# Autodesk Inventor assembly: Table
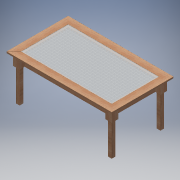
[picture p0: Inventor's stored thumbnail of the model, 180x180]
Saved by Autodesk Inventor 2016 (Build 200138000, 138)
## iProperties
Created: 2016-02-08
Part Number: Table
Document SubType Name: Assembly
Designer: ron
Mass: 50986 g
Surface Area: 141310 cm^2
Volume: 60602.2 cm^3
Density: 0.841322 g/cm^3
Author: ron
## Documents named in this file (20)
- C:\Users\ron\Documents\GitHub\CoffeeTableCAD\Table.iam
- C:\Users\ron\Documents\GitHub\CoffeeTableCAD\Parts\LedBoard.ipt
- C:\Users\ron\Documents\GitHub\CoffeeTableCAD\Parts\Acrylitep95.ipt
- C:\Users\ron\Documents\GitHub\CoffeeTableCAD\Parts\LegStandard.ipt
- C:\Users\ron\Documents\GitHub\CoffeeTableCAD\Parts\Glass.ipt
- C:\Users\ron\Documents\GitHub\CoffeeTableCAD\Parts\LegOutlet.ipt
- C:\Users\ron\Documents\GitHub\CoffeeTableCAD\Parts\Bottom.ipt
- C:\Users\ron\Documents\GitHub\CoffeeTableCAD\Parts\PowerSupply.ipt
- C:\Users\ron\Documents\GitHub\CoffeeTableCAD\Parts\Magnet.ipt
- C:\Users\ron\Documents\GitHub\CoffeeTableCAD\Parts\DividerWidthPlastic.ipt
- C:\Users\ron\Documents\GitHub\CoffeeTableCAD\Parts\DividerLengthPlastic.ipt
- C:\Users\ron\Documents\GitHub\CoffeeTableCAD\Parts\SkinnySideWidth.ipt
- C:\Users\ron\Documents\GitHub\CoffeeTableCAD\Parts\SkinnySideLength.ipt
- C:\Users\ron\Documents\GitHub\CoffeeTableCAD\Parts\SkirtLength.ipt
- C:\Users\ron\Documents\GitHub\CoffeeTableCAD\Parts\SkirtWidth.ipt
- C:\Users\ron\Documents\GitHub\CoffeeTableCAD\Parts\LegHolder.ipt
- C:\Users\ron\Documents\GitHub\CoffeeTableCAD\Parts\SkinnySideWidthOutlet.ipt
- C:\Users\ron\Documents\GitHub\CoffeeTableCAD\Parts\SkinnySideLengthPower.ipt
- C:\Users\ron\Documents\GitHub\CoffeeTableCAD\Parts\LegHolderOutlet.ipt
- C:\Users\ron\Documents\GitHub\CoffeeTableCAD\Parts\SupportWedge.ipt
## Components (77 placed, 19 different names)
1. LedBoard:1 — Flush:127, Flush:128, Mate:93, Mate:94, Flush:138, Flush:139, Flush:140, Flush:141, Flush:143, Flush:144, Flush:146, Flush:147, Flush:149, Flush:150, Flush:152, Flush:153, Flush:155, Flush:156, Flush:158, Flush:159, Flush:161, Flush:162, Flush:164, Flush:165, Flush:167, Flush:168, Flush:170, Flush:171, Flush:173, Flush:174, Flush:176, Flush:177, Flush:179, Flush:180, Flush:182, Flush:183, Flush:185, Flush:186, Flush:188, Flush:189, Flush:191, Flush:192, Flush:194, Flush:195, Flush:197, Flush:198, Flush:200, Flush:201, Flush:203, Flush:204, Flush:206, Flush:207, Flush:209, Flush:210, Flush:212, Flush:213, Flush:215, Flush:216, Flush:218, Flush:220, Flush:221, Flush:223, Flush:224, Flush:226, Flush:227, Flush:229, Mate:95, Flush:230, Flush:231, Mate:96, Flush:232, Mate:97, Flush:234, Mate:98, Flush:236, Mate:99, Flush:238, Mate:100, Flush:240, Mate:101, Flush:242, Mate:102, Flush:244, Mate:103, Flush:246, Mate:104, Flush:249, Mate:105, Flush:251, Mate:106, Flush:253, Mate:107, Flush:255, Mate:108, Flush:257, Mate:109, Flush:259, Mate:113, Mate:115, Mate:128, Mate:129, Mate:130, Mate:131, Mate:139, Mate:142, Mate:144
2. Acrylitep95:1 — Flush:127, Flush:128, Mate:20, Flush:129, Flush:130, Mate:93, Mate:117, Mate:119, Mate:122, Mate:125
3. LegStandard:1 — Mate:89, Mate:90, Flush:136, Mate:135, Mate:136, Mate:137
4. LegStandard:2 — Mate:91, Mate:92, Flush:137, Mate:148, Mate:149, Mate:150
5. LegStandard:3 — Mate:85, Mate:86, Flush:134, Mate:151, Mate:152, Mate:153
6. LegOutlet:1 — Mate:87, Mate:88, Flush:135, Mate:138, Mate:145, Mate:146, Mate:147
7. Glass:1 — Mate:20, Flush:129, Flush:130, Mate:118, Mate:121, Mate:124
8. Bottom:1 — Flush:131, Flush:132, Mate:167, Mate:168, Mate:169, Mate:170
9. PowerSupply:1 — Flush:131, Flush:132, Mate:170
10. Magnet:3 — Mate:85, Mate:86, Flush:134
11. Magnet:4 — Mate:89, Mate:90, Flush:136
12. Magnet:5 — Mate:87, Mate:88, Flush:135
13. Magnet:6 — Mate:91, Mate:92, Flush:137
14. DividerWidthPlastic:1 — Flush:161, Flush:162, Flush:163, Flush:166
15. DividerWidthPlastic:2 — Flush:167, Flush:168, Flush:169, Flush:172
16. DividerWidthPlastic:3 — Flush:176, Flush:177, Flush:178, Flush:181
17. DividerWidthPlastic:4 — Flush:215, Flush:216, Flush:217, Flush:219
18. DividerWidthPlastic:6 — Flush:170, Flush:171, Flush:172, Flush:175
19. DividerWidthPlastic:7 — Flush:164, Flush:165, Flush:166, Flush:169
20. DividerWidthPlastic:8 — Flush:155, Flush:156, Flush:157, Flush:160
21. DividerWidthPlastic:9 — Flush:158, Flush:159, Flush:160, Flush:163
22. DividerWidthPlastic:10 — Flush:188, Flush:189, Flush:190, Flush:193
23. DividerWidthPlastic:11 — Flush:212, Flush:213, Flush:214, Flush:217
24. DividerWidthPlastic:12 — Flush:218, Flush:219, Flush:220, Flush:222
25. DividerWidthPlastic:13 — Flush:185, Flush:186, Flush:187, Flush:190
26. DividerWidthPlastic:14 — Flush:182, Flush:183, Flush:184, Flush:187
27. DividerWidthPlastic:15 — Flush:179, Flush:180, Flush:181, Flush:184
28. DividerWidthPlastic:16 — Flush:200, Flush:201, Flush:202, Flush:205
29. DividerWidthPlastic:17 — Flush:194, Flush:195, Flush:196, Flush:199
30. DividerWidthPlastic:18 — Flush:191, Flush:192, Flush:193, Flush:196
31. DividerWidthPlastic:19 — Flush:197, Flush:198, Flush:199, Flush:202
32. DividerWidthPlastic:20 — Flush:209, Flush:210, Flush:211, Flush:214
33. DividerWidthPlastic:21 — Mate:94, Flush:138, Flush:139, Flush:142
34. DividerWidthPlastic:22 — Flush:149, Flush:150, Flush:151, Flush:154
35. DividerWidthPlastic:23 — Flush:206, Flush:207, Flush:208, Flush:211
36. DividerWidthPlastic:24 — Flush:140, Flush:141, Flush:142, Flush:145, Mate:120
37. DividerWidthPlastic:25 — Flush:203, Flush:204, Flush:205, Flush:208
38. DividerWidthPlastic:26 — Flush:143, Flush:144, Flush:145, Flush:148
39. DividerWidthPlastic:27 — Flush:146, Flush:147, Flush:148, Flush:151
40. DividerWidthPlastic:28 — Flush:152, Flush:153, Flush:154, Flush:157
41. DividerWidthPlastic:29 — Flush:221, Flush:222, Flush:223, Flush:225
42. DividerWidthPlastic:30 — Flush:224, Flush:225, Flush:226, Flush:228
43. DividerWidthPlastic:31 — Flush:227, Flush:228, Flush:229
44. DividerWidthPlastic:32 — Flush:173, Flush:174, Flush:175, Flush:178
45. DividerLengthPlastic:1 — Mate:95, Flush:230, Flush:231, Flush:233
46. DividerLengthPlastic:2 — Mate:98, Flush:236, Flush:237, Flush:239
47. DividerLengthPlastic:3 — Mate:99, Flush:238, Flush:239, Flush:241
48. DividerLengthPlastic:4 — Mate:104, Flush:248, Flush:249, Flush:250
49. DividerLengthPlastic:5 — Mate:107, Flush:254, Flush:255, Flush:256
50. DividerLengthPlastic:7 — Mate:109, Flush:258, Flush:259
51. DividerLengthPlastic:8 — Mate:105, Flush:250, Flush:251, Flush:252
52. DividerLengthPlastic:9 — Mate:103, Flush:246, Flush:247, Flush:248
53. DividerLengthPlastic:10 — Mate:101, Flush:242, Flush:243, Flush:245
54. DividerLengthPlastic:11 — Mate:97, Flush:234, Flush:235, Flush:237
55. DividerLengthPlastic:12 — Mate:96, Flush:232, Flush:233, Flush:235
56. DividerLengthPlastic:13 — Mate:100, Flush:240, Flush:241, Flush:243, Mate:141
57. DividerLengthPlastic:14 — Mate:102, Flush:244, Flush:245, Flush:247
58. DividerLengthPlastic:15 — Mate:106, Flush:252, Flush:253, Flush:254, Mate:123
59. DividerLengthPlastic:17 — Mate:108, Flush:256, Flush:257, Flush:258, Mate:116
60. SkinnySideWidth:1 — Mate:113, Mate:115, Mate:128, Mate:134, Mate:143, Mate:152, Mate:156, Flush:260, Flush:261, Mate:167, Mate:169
61. SkirtLength:1 — Mate:119, Mate:120, Mate:121, Mate:132, Mate:148, Mate:171, Mate:180, Mate:181, Mate:182
62. SkirtLength:2 — Mate:125, Mate:126, Mate:127, Mate:151, Mate:154, Mate:174, Mate:175, Mate:177, Mate:179
63. SkirtWidth:1 — Mate:116, Mate:117, Mate:118, Mate:127, Mate:135, Mate:176
64. SkirtWidth:2 — Mate:122, Mate:123, Mate:124, Mate:126, Mate:138, Mate:145, Mate:147, Mate:150, Mate:157, Mate:160, Mate:172, Mate:173, Mate:178
65. SkinnySideLength:1 — Mate:129, Mate:130, Mate:131, Mate:133, Mate:140, Mate:149, Mate:159, Mate:166
66. SkinnySideWidthOutlet:1 — Mate:139, Mate:140, Mate:141, Mate:158, Mate:162, Mate:164, Mate:165
67. SkinnySideLengthPower:1 — Mate:142, Mate:143, Mate:144, Mate:146, Mate:153, Mate:155, Mate:161, Mate:163, Mate:168
68. LegHolder:1 — Mate:132, Mate:133, Mate:134, Mate:136, Mate:137
69. LegHolder:2 — Mate:154, Mate:155, Mate:156
70. LegHolder:3 — Mate:157, Mate:158, Mate:159
71. LegHolderOutlet:1 — Mate:160, Mate:161, Mate:162
72. SupportWedge:1 — Flush:260, Mate:163, Mate:164
73. SupportWedge:2 — Flush:261, Mate:165, Mate:166
74. Magnet:7 — Mate:180, Mate:181, Mate:182
75. Magnet:8 — Mate:174, Mate:175, Mate:176
76. Magnet:9 — Mate:171, Mate:172, Mate:173
77. Magnet:10 — Mate:177, Mate:178, Mate:179
## Relationships (229: Flush 134, Mate 95)
- Flush:127 (-25.4 mm): LedBoard:1 ↔ Acrylitep95:1
- Flush:128 (-25.4 mm): LedBoard:1 ↔ Acrylitep95:1
- Mate:20: Acrylitep95:1 ↔ Glass:1
- Flush:129: Acrylitep95:1 ↔ Glass:1
- Flush:130: Acrylitep95:1 ↔ Glass:1
- Flush:131 (50.8 mm): Bottom:1 ↔ PowerSupply:1
- Flush:132 (50.8 mm): Bottom:1 ↔ PowerSupply:1
- Mate:85: LegStandard:3 ↔ Magnet:3
- Mate:86: LegStandard:3 ↔ Magnet:3
- Flush:134: LegStandard:3 ↔ Magnet:3
- Mate:87: LegOutlet:1 ↔ Magnet:5
- Mate:88: LegOutlet:1 ↔ Magnet:5
- Flush:135: LegOutlet:1 ↔ Magnet:5
- Mate:89: LegStandard:1 ↔ Magnet:4
- Mate:90: LegStandard:1 ↔ Magnet:4
- Flush:136: LegStandard:1 ↔ Magnet:4
- Mate:91: LegStandard:2 ↔ Magnet:6
- Mate:92: LegStandard:2 ↔ Magnet:6
- Flush:137: LegStandard:2 ↔ Magnet:6
- Mate:93 (50.8 mm): LedBoard:1 ↔ Acrylitep95:1
- Mate:94: LedBoard:1 ↔ DividerWidthPlastic:21
- Flush:138: LedBoard:1 ↔ DividerWidthPlastic:21
- Flush:139 (36.5125 mm): LedBoard:1 ↔ DividerWidthPlastic:21
- Flush:140 (-50.8 mm): LedBoard:1 ↔ DividerWidthPlastic:24
- Flush:141: LedBoard:1 ↔ DividerWidthPlastic:24
- Flush:142 (38.1 mm): DividerWidthPlastic:21 ↔ DividerWidthPlastic:24
- Flush:143 (-50.8 mm): LedBoard:1 ↔ DividerWidthPlastic:26
- Flush:144: LedBoard:1 ↔ DividerWidthPlastic:26
- Flush:145 (38.1 mm): DividerWidthPlastic:24 ↔ DividerWidthPlastic:26
- Flush:146 (-50.8 mm): LedBoard:1 ↔ DividerWidthPlastic:27
- Flush:147: LedBoard:1 ↔ DividerWidthPlastic:27
- Flush:148 (38.1 mm): DividerWidthPlastic:26 ↔ DividerWidthPlastic:27
- Flush:149 (-50.8 mm): LedBoard:1 ↔ DividerWidthPlastic:22
- Flush:150: LedBoard:1 ↔ DividerWidthPlastic:22
- Flush:151 (38.1 mm): DividerWidthPlastic:22 ↔ DividerWidthPlastic:27
- Flush:152 (-50.8 mm): LedBoard:1 ↔ DividerWidthPlastic:28
- Flush:153: LedBoard:1 ↔ DividerWidthPlastic:28
- Flush:154 (38.1 mm): DividerWidthPlastic:22 ↔ DividerWidthPlastic:28
- Flush:155 (-50.8 mm): LedBoard:1 ↔ DividerWidthPlastic:8
- Flush:156: LedBoard:1 ↔ DividerWidthPlastic:8
- Flush:157 (38.1 mm): DividerWidthPlastic:8 ↔ DividerWidthPlastic:28
- Flush:158 (-50.8 mm): LedBoard:1 ↔ DividerWidthPlastic:9
- Flush:159: LedBoard:1 ↔ DividerWidthPlastic:9
- Flush:160 (38.1 mm): DividerWidthPlastic:8 ↔ DividerWidthPlastic:9
- Flush:161 (-50.8 mm): LedBoard:1 ↔ DividerWidthPlastic:1
- Flush:162: LedBoard:1 ↔ DividerWidthPlastic:1
- Flush:163 (38.1 mm): DividerWidthPlastic:1 ↔ DividerWidthPlastic:9
- Flush:164 (-50.8 mm): LedBoard:1 ↔ DividerWidthPlastic:7
- Flush:165: LedBoard:1 ↔ DividerWidthPlastic:7
- Flush:166 (38.1 mm): DividerWidthPlastic:1 ↔ DividerWidthPlastic:7
- Flush:167 (-50.8 mm): LedBoard:1 ↔ DividerWidthPlastic:2
- Flush:168: LedBoard:1 ↔ DividerWidthPlastic:2
- Flush:169 (38.1 mm): DividerWidthPlastic:2 ↔ DividerWidthPlastic:7
- Flush:170 (-50.8 mm): LedBoard:1 ↔ DividerWidthPlastic:6
- Flush:171: LedBoard:1 ↔ DividerWidthPlastic:6
- Flush:172 (38.1 mm): DividerWidthPlastic:2 ↔ DividerWidthPlastic:6
- Flush:173 (-50.8 mm): LedBoard:1 ↔ DividerWidthPlastic:32
- Flush:174: LedBoard:1 ↔ DividerWidthPlastic:32
- Flush:175 (38.1 mm): DividerWidthPlastic:6 ↔ DividerWidthPlastic:32
- Flush:176 (-50.8 mm): LedBoard:1 ↔ DividerWidthPlastic:3
- Flush:177: LedBoard:1 ↔ DividerWidthPlastic:3
- Flush:178 (38.1 mm): DividerWidthPlastic:3 ↔ DividerWidthPlastic:32
- Flush:179 (-50.8 mm): LedBoard:1 ↔ DividerWidthPlastic:15
- Flush:180: LedBoard:1 ↔ DividerWidthPlastic:15
- Flush:181 (38.1 mm): DividerWidthPlastic:3 ↔ DividerWidthPlastic:15
- Flush:182 (-50.8 mm): LedBoard:1 ↔ DividerWidthPlastic:14
- Flush:183: LedBoard:1 ↔ DividerWidthPlastic:14
- Flush:184 (38.1 mm): DividerWidthPlastic:14 ↔ DividerWidthPlastic:15
- Flush:185 (-50.8 mm): LedBoard:1 ↔ DividerWidthPlastic:13
- Flush:186: LedBoard:1 ↔ DividerWidthPlastic:13
- Flush:187 (38.1 mm): DividerWidthPlastic:13 ↔ DividerWidthPlastic:14
- Flush:188 (-50.8 mm): LedBoard:1 ↔ DividerWidthPlastic:10
- Flush:189: LedBoard:1 ↔ DividerWidthPlastic:10
- Flush:190 (38.1 mm): DividerWidthPlastic:10 ↔ DividerWidthPlastic:13
- Flush:191 (-50.8 mm): LedBoard:1 ↔ DividerWidthPlastic:18
- Flush:192: LedBoard:1 ↔ DividerWidthPlastic:18
- Flush:193 (38.1 mm): DividerWidthPlastic:10 ↔ DividerWidthPlastic:18
- Flush:194 (-50.8 mm): LedBoard:1 ↔ DividerWidthPlastic:17
- Flush:195: LedBoard:1 ↔ DividerWidthPlastic:17
- Flush:196 (38.1 mm): DividerWidthPlastic:17 ↔ DividerWidthPlastic:18
- Flush:197 (-50.8 mm): LedBoard:1 ↔ DividerWidthPlastic:19
- Flush:198: LedBoard:1 ↔ DividerWidthPlastic:19
- Flush:199 (38.1 mm): DividerWidthPlastic:17 ↔ DividerWidthPlastic:19
- Flush:200 (-50.8 mm): LedBoard:1 ↔ DividerWidthPlastic:16
- Flush:201: LedBoard:1 ↔ DividerWidthPlastic:16
- Flush:202 (38.1 mm): DividerWidthPlastic:16 ↔ DividerWidthPlastic:19
- Flush:203 (-50.8 mm): LedBoard:1 ↔ DividerWidthPlastic:25
- Flush:204: LedBoard:1 ↔ DividerWidthPlastic:25
- Flush:205 (38.1 mm): DividerWidthPlastic:16 ↔ DividerWidthPlastic:25
- Flush:206 (-50.8 mm): LedBoard:1 ↔ DividerWidthPlastic:23
- Flush:207: LedBoard:1 ↔ DividerWidthPlastic:23
- Flush:208 (38.1 mm): DividerWidthPlastic:23 ↔ DividerWidthPlastic:25
- Flush:209 (-50.8 mm): LedBoard:1 ↔ DividerWidthPlastic:20
- Flush:210: LedBoard:1 ↔ DividerWidthPlastic:20
- Flush:211 (38.1 mm): DividerWidthPlastic:20 ↔ DividerWidthPlastic:23
- Flush:212 (-50.8 mm): LedBoard:1 ↔ DividerWidthPlastic:11
- Flush:213: LedBoard:1 ↔ DividerWidthPlastic:11
- Flush:214 (38.1 mm): DividerWidthPlastic:11 ↔ DividerWidthPlastic:20
- Flush:215 (-50.8 mm): LedBoard:1 ↔ DividerWidthPlastic:4
- Flush:216: LedBoard:1 ↔ DividerWidthPlastic:4
- Flush:217 (38.1 mm): DividerWidthPlastic:4 ↔ DividerWidthPlastic:11
- Flush:218 (-50.8 mm): LedBoard:1 ↔ DividerWidthPlastic:12
- Flush:219 (38.1 mm): DividerWidthPlastic:4 ↔ DividerWidthPlastic:12
- Flush:220: LedBoard:1 ↔ DividerWidthPlastic:12
- Flush:221 (-50.8 mm): LedBoard:1 ↔ DividerWidthPlastic:29
- Flush:222 (38.1 mm): DividerWidthPlastic:12 ↔ DividerWidthPlastic:29
- Flush:223: LedBoard:1 ↔ DividerWidthPlastic:29
- Flush:224 (-50.8 mm): LedBoard:1 ↔ DividerWidthPlastic:30
- Flush:225 (38.1 mm): DividerWidthPlastic:29 ↔ DividerWidthPlastic:30
- Flush:226: LedBoard:1 ↔ DividerWidthPlastic:30
- Flush:227 (-50.8 mm): LedBoard:1 ↔ DividerWidthPlastic:31
- Flush:228 (38.1 mm): DividerWidthPlastic:30 ↔ DividerWidthPlastic:31
- Flush:229: LedBoard:1 ↔ DividerWidthPlastic:31
- Mate:95: LedBoard:1 ↔ DividerLengthPlastic:1
- Flush:230: LedBoard:1 ↔ DividerLengthPlastic:1
- Flush:231 (36.5125 mm): LedBoard:1 ↔ DividerLengthPlastic:1
- Mate:96: LedBoard:1 ↔ DividerLengthPlastic:12
- Flush:232: LedBoard:1 ↔ DividerLengthPlastic:12
- Flush:233 (-38.1 mm): DividerLengthPlastic:1 ↔ DividerLengthPlastic:12
- Mate:97: LedBoard:1 ↔ DividerLengthPlastic:11
- Flush:234: LedBoard:1 ↔ DividerLengthPlastic:11
- Flush:235 (38.1 mm): DividerLengthPlastic:11 ↔ DividerLengthPlastic:12
- Mate:98: LedBoard:1 ↔ DividerLengthPlastic:2
- Flush:236: LedBoard:1 ↔ DividerLengthPlastic:2
- Flush:237 (38.1 mm): DividerLengthPlastic:2 ↔ DividerLengthPlastic:11
- Mate:99: LedBoard:1 ↔ DividerLengthPlastic:3
- Flush:238: LedBoard:1 ↔ DividerLengthPlastic:3
- Flush:239 (38.1 mm): DividerLengthPlastic:2 ↔ DividerLengthPlastic:3
- Mate:100: LedBoard:1 ↔ DividerLengthPlastic:13
- Flush:240: LedBoard:1 ↔ DividerLengthPlastic:13
- Flush:241 (38.1 mm): DividerLengthPlastic:3 ↔ DividerLengthPlastic:13
- Mate:101: LedBoard:1 ↔ DividerLengthPlastic:10
- Flush:242: LedBoard:1 ↔ DividerLengthPlastic:10
- Flush:243 (38.1 mm): DividerLengthPlastic:10 ↔ DividerLengthPlastic:13
- Mate:102: LedBoard:1 ↔ DividerLengthPlastic:14
- Flush:244: LedBoard:1 ↔ DividerLengthPlastic:14
- Flush:245 (38.1 mm): DividerLengthPlastic:10 ↔ DividerLengthPlastic:14
- Mate:103: LedBoard:1 ↔ DividerLengthPlastic:9
- Flush:246: LedBoard:1 ↔ DividerLengthPlastic:9
- Flush:247 (38.1 mm): DividerLengthPlastic:9 ↔ DividerLengthPlastic:14
- Mate:104: LedBoard:1 ↔ DividerLengthPlastic:4
- Flush:248 (38.1 mm): DividerLengthPlastic:4 ↔ DividerLengthPlastic:9
- Flush:249: LedBoard:1 ↔ DividerLengthPlastic:4
- Mate:105: LedBoard:1 ↔ DividerLengthPlastic:8
- Flush:250 (38.1 mm): DividerLengthPlastic:4 ↔ DividerLengthPlastic:8
- Flush:251: LedBoard:1 ↔ DividerLengthPlastic:8
- Mate:106: LedBoard:1 ↔ DividerLengthPlastic:15
- Flush:252 (38.1 mm): DividerLengthPlastic:8 ↔ DividerLengthPlastic:15
- Flush:253: LedBoard:1 ↔ DividerLengthPlastic:15
- Mate:107: LedBoard:1 ↔ DividerLengthPlastic:5
- Flush:254 (38.1 mm): DividerLengthPlastic:5 ↔ DividerLengthPlastic:15
- Flush:255: LedBoard:1 ↔ DividerLengthPlastic:5
- Mate:108: LedBoard:1 ↔ DividerLengthPlastic:17
- Flush:256 (38.1 mm): DividerLengthPlastic:5 ↔ DividerLengthPlastic:17
- Flush:257: LedBoard:1 ↔ DividerLengthPlastic:17
- Mate:109: LedBoard:1 ↔ DividerLengthPlastic:7
- Flush:258 (38.1 mm): DividerLengthPlastic:7 ↔ DividerLengthPlastic:17
- Flush:259: LedBoard:1 ↔ DividerLengthPlastic:7
- Mate:113: LedBoard:1 ↔ SkinnySideWidth:1
- Mate:115: LedBoard:1 ↔ SkinnySideWidth:1
- Mate:116: DividerLengthPlastic:17 ↔ SkirtWidth:1
- Mate:117: Acrylitep95:1 ↔ SkirtWidth:1
- Mate:118: Glass:1 ↔ SkirtWidth:1
- Mate:119: Acrylitep95:1 ↔ SkirtLength:1
- Mate:120: DividerWidthPlastic:24 ↔ SkirtLength:1
- Mate:121: Glass:1 ↔ SkirtLength:1
- Mate:122: Acrylitep95:1 ↔ SkirtWidth:2
- Mate:123: DividerLengthPlastic:15 ↔ SkirtWidth:2
- Mate:124: Glass:1 ↔ SkirtWidth:2
- Mate:125: Acrylitep95:1 ↔ SkirtLength:2
- Mate:126: SkirtLength:2 ↔ SkirtWidth:2
- Mate:127: SkirtLength:2 ↔ SkirtWidth:1
- Mate:128: LedBoard:1 ↔ SkinnySideWidth:1
- Mate:129: LedBoard:1 ↔ SkinnySideLength:1
- Mate:130: LedBoard:1 ↔ SkinnySideLength:1
- Mate:131: LedBoard:1 ↔ SkinnySideLength:1
- Mate:132: SkirtLength:1 ↔ LegHolder:1
- Mate:133: SkinnySideLength:1 ↔ LegHolder:1
- Mate:134: SkinnySideWidth:1 ↔ LegHolder:1
- Mate:135: LegStandard:1 ↔ SkirtWidth:1
- Mate:136: LegStandard:1 ↔ LegHolder:1
- Mate:137: LegStandard:1 ↔ LegHolder:1
- Mate:138: LegOutlet:1 ↔ SkirtWidth:2
- Mate:139: LedBoard:1 ↔ SkinnySideWidthOutlet:1
- Mate:140: SkinnySideLength:1 ↔ SkinnySideWidthOutlet:1
- Mate:141: DividerLengthPlastic:13 ↔ SkinnySideWidthOutlet:1
- Mate:142: LedBoard:1 ↔ SkinnySideLengthPower:1
- Mate:143: SkinnySideWidth:1 ↔ SkinnySideLengthPower:1
- Mate:144: LedBoard:1 ↔ SkinnySideLengthPower:1
- Mate:145: LegOutlet:1 ↔ SkirtWidth:2
- Mate:146: LegOutlet:1 ↔ SkinnySideLengthPower:1
- Mate:147 (-117.1702 mm): LegOutlet:1 ↔ SkirtWidth:2
- Mate:148: LegStandard:2 ↔ SkirtLength:1
- Mate:149: LegStandard:2 ↔ SkinnySideLength:1
- Mate:150 (-117.1702 mm): LegStandard:2 ↔ SkirtWidth:2
- Mate:151: LegStandard:3 ↔ SkirtLength:2
- Mate:152: LegStandard:3 ↔ SkinnySideWidth:1
- Mate:153: LegStandard:3 ↔ SkinnySideLengthPower:1
- Mate:154: SkirtLength:2 ↔ LegHolder:2
- Mate:155: SkinnySideLengthPower:1 ↔ LegHolder:2
- Mate:156: SkinnySideWidth:1 ↔ LegHolder:2
- Mate:157: SkirtWidth:2 ↔ LegHolder:3
- Mate:158: SkinnySideWidthOutlet:1 ↔ LegHolder:3
- Mate:159: SkinnySideLength:1 ↔ LegHolder:3
- Mate:160: SkirtWidth:2 ↔ LegHolderOutlet:1
- Mate:161: SkinnySideLengthPower:1 ↔ LegHolderOutlet:1
- Mate:162: SkinnySideWidthOutlet:1 ↔ LegHolderOutlet:1
- Flush:260: SkinnySideWidth:1 ↔ SupportWedge:1
- Mate:163: SkinnySideLengthPower:1 ↔ SupportWedge:1
- Mate:164: SkinnySideWidthOutlet:1 ↔ SupportWedge:1
- Flush:261: SkinnySideWidth:1 ↔ SupportWedge:2
- Mate:165: SkinnySideWidthOutlet:1 ↔ SupportWedge:2
- Mate:166: SkinnySideLength:1 ↔ SupportWedge:2
- Mate:167: Bottom:1 ↔ SkinnySideWidth:1
- Mate:168: Bottom:1 ↔ SkinnySideLengthPower:1
- Mate:169: Bottom:1 ↔ SkinnySideWidth:1
- Mate:170: Bottom:1 ↔ PowerSupply:1
- Mate:171: SkirtLength:1 ↔ Magnet:9
- Mate:172: SkirtWidth:2 ↔ Magnet:9
- Mate:173: SkirtWidth:2 ↔ Magnet:9
- Mate:174: SkirtLength:2 ↔ Magnet:8
- Mate:175: SkirtLength:2 ↔ Magnet:8
- Mate:176: SkirtWidth:1 ↔ Magnet:8
- Mate:177: SkirtLength:2 ↔ Magnet:10
- Mate:178: SkirtWidth:2 ↔ Magnet:10
- Mate:179: SkirtLength:2 ↔ Magnet:10
- Mate:180: SkirtLength:1 ↔ Magnet:7
- Mate:181: SkirtLength:1 ↔ Magnet:7
- Mate:182: SkirtLength:1 ↔ Magnet:7
